# Autodesk Inventor assembly: ASY PRS 1610 charging hatch_D1200
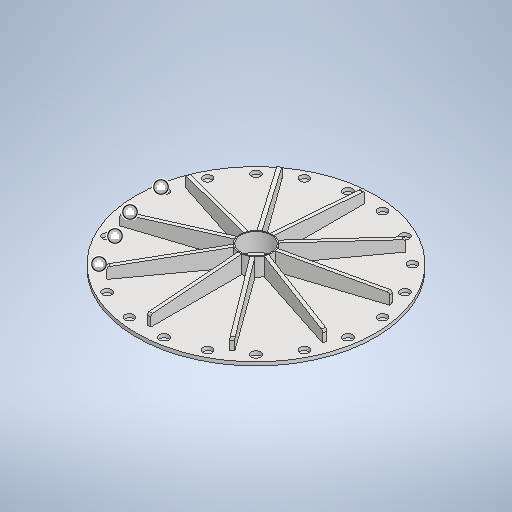
[picture p0: Inventor's stored thumbnail of the model, 512x512]
Saved by Autodesk Inventor 2026.2 (Build 302298000, 298)
## iProperties
Created: 2025-04-22
Part Number: ASY PRS 1610 charging hatch_D1200
Document SubType Name: Assembly
Designer: admin
Mass: 9483.1 g
Surface Area: 9977.57 cm^2
Volume: 3616.18 cm^3
Density: 2.6224 g/cm^3
Author: user
## Documents named in this file (4)
- C:\Users\admin\Documents\Inventor\PRS-Purovsk\ASY PRS 1610 charging hatch_D1200.iam
- C:\Users\admin\Documents\Inventor\PRS-Purovsk\PRS 1621 charging hatch D1200.ipt
- C:\Users\admin\Documents\Inventor\PRS-Purovsk\PRS 1611 hatch tube 500mm_D1200.ipt
- C:\Users\admin\Documents\Inventor\PRS-Purovsk\PRS 1614 charging hatch reinf 500mm_D1200.ipt
## Components (12 placed, 3 different names)
1. PRS 1621 charging hatch D1200:1 — Rigid:1, Mate:1
2. PRS 1611 hatch tube 500mm_D1200:1 — Rigid:1, Tangent:1
3. PRS 1614 charging hatch reinf 500mm_D1200:1 — Mate:1, Mate:2, Tangent:1
4. PRS 1614 charging hatch reinf 500mm_D1200:2
5. PRS 1614 charging hatch reinf 500mm_D1200:3
6. PRS 1614 charging hatch reinf 500mm_D1200:4
7. PRS 1614 charging hatch reinf 500mm_D1200:5
8. PRS 1614 charging hatch reinf 500mm_D1200:6
9. PRS 1614 charging hatch reinf 500mm_D1200:7
10. PRS 1614 charging hatch reinf 500mm_D1200:8
11. PRS 1614 charging hatch reinf 500mm_D1200:9
12. PRS 1614 charging hatch reinf 500mm_D1200:10
## Component patterns: (10 elements, first: PRS 1614 charging hatch reinf 500mm_D1200:1)
## Relationships (4: Mate 2, WeldJoint 1, Tangent 1)
- Rigid:1 [WeldJoint]: PRS 1621 charging hatch D1200:1 ↔ PRS 1611 hatch tube 500mm_D1200:1
- Mate:1: PRS 1621 charging hatch D1200:1 ↔ PRS 1614 charging hatch reinf 500mm_D1200:1
- Mate:2: PRS 1614 charging hatch reinf 500mm_D1200:1
- Tangent:1: PRS 1611 hatch tube 500mm_D1200:1 ↔ PRS 1614 charging hatch reinf 500mm_D1200:1
